# Autodesk Inventor assembly: Slider Assembly
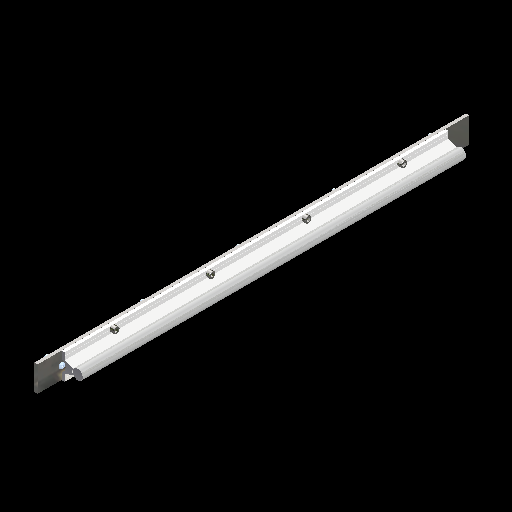
[picture p0: Inventor's stored thumbnail of the model, 512x512]
Saved by Autodesk Inventor 2026.1 (Build 301233000, 233)
## iProperties
Created: 2024-12-30
Part Number: Slider Assembly
Document SubType Name: Assembly
Designer: drago
Author: drago
## Documents named in this file (5)
- C:\Users\drago\Desktop\_QIST4500_Multidisciplinary_Team_Project\Proteox MX magnet positioner CAD\z_rail\z_rail.iam
- C:\Users\drago\Desktop\_QIST4500_Multidisciplinary_Team_Project\Proteox MX magnet positioner CAD\z_rail\item_61953_t-slot-slider-8-80x40-fa__high.ipt
- C:\Users\drago\Desktop\_QIST4500_Multidisciplinary_Team_Project\Proteox MX magnet positioner CAD\z_rail\Rail_bracket.ipt
- C:\Users\drago\Desktop\_QIST4500_Multidisciplinary_Team_Project\Proteox MX magnet positioner CAD\z_rail\SBR16_600mm.ipt
- C:\Users\drago\Documents\Inventor\Content Center Files\R2026\en-US\ISO 4762(2)\ISO 4762 - M6 x 10ISO.ipt
## Components (15 placed, 4 different names)
1. Rail_bracket:1 — Mate:15, Mate:16, Mate:17, Mate:18, Mate:19, Mate:20, Mate:21, Mate:22, Mate:23, Mate:24, Mate:25, Mate:26, Mate:27, Mate:28, Mate:29, Mate:36, Mate:38, Mate:40, Mate:42, Mate:44, Mate:46, Mate:48, Mate:50
2. SBR16_600mm:1 — Mate:16, Mate:17, Mate:18, Mate:37, Mate:39, Mate:41, Mate:43, Mate:45, Mate:47, Mate:49, Mate:51
3. item_61953_t-slot-slider-8-80x40-fa__high:1 — Mate:20, Mate:21, Angle:1
4. item_61953_t-slot-slider-8-80x40-fa__high:2 — Mate:24, Mate:28, Angle:2
5. item_61953_t-slot-slider-8-80x40-fa__high:3 — Mate:22, Mate:26, Angle:3
6. item_61953_t-slot-slider-8-80x40-fa__high:4 — Mate:23, Mate:27, Angle:4
7. item_61953_t-slot-slider-8-80x40-fa__high:5 — Mate:25, Mate:29, Angle:5
8. ISO 4762 M6 x 10:1 — Mate:36, Mate:37
9. ISO 4762 M6 x 10:2 — Mate:38, Mate:39
10. ISO 4762 M6 x 10:3 — Mate:40, Mate:41
11. ISO 4762 M6 x 10:4 — Mate:42, Mate:43
12. ISO 4762 M6 x 10:5 — Mate:44, Mate:45
13. ISO 4762 M6 x 10:6 — Mate:46, Mate:47
14. ISO 4762 M6 x 10:7 — Mate:48, Mate:49
15. ISO 4762 M6 x 10:8 — Mate:50, Mate:51
## Relationships (36: Mate 31, Angle 5)
- Mate:15: Rail_bracket:1
- Mate:16: Rail_bracket:1 ↔ SBR16_600mm:1
- Mate:17: Rail_bracket:1 ↔ SBR16_600mm:1
- Mate:18: Rail_bracket:1 ↔ SBR16_600mm:1
- Mate:19: Rail_bracket:1
- Mate:20: Rail_bracket:1 ↔ item_61953_t-slot-slider-8-80x40-fa__high:1
- Mate:21: Rail_bracket:1 ↔ item_61953_t-slot-slider-8-80x40-fa__high:1
- Angle:1 (0 deg): item_61953_t-slot-slider-8-80x40-fa__high:1
- Mate:22: Rail_bracket:1 ↔ item_61953_t-slot-slider-8-80x40-fa__high:3
- Mate:23: Rail_bracket:1 ↔ item_61953_t-slot-slider-8-80x40-fa__high:4
- Mate:24: Rail_bracket:1 ↔ item_61953_t-slot-slider-8-80x40-fa__high:2
- Mate:25: Rail_bracket:1 ↔ item_61953_t-slot-slider-8-80x40-fa__high:5
- Mate:26: Rail_bracket:1 ↔ item_61953_t-slot-slider-8-80x40-fa__high:3
- Mate:27: Rail_bracket:1 ↔ item_61953_t-slot-slider-8-80x40-fa__high:4
- Mate:28: Rail_bracket:1 ↔ item_61953_t-slot-slider-8-80x40-fa__high:2
- Mate:29: Rail_bracket:1 ↔ item_61953_t-slot-slider-8-80x40-fa__high:5
- Angle:2 (0 deg): item_61953_t-slot-slider-8-80x40-fa__high:2
- Angle:3 (0 deg): item_61953_t-slot-slider-8-80x40-fa__high:3
- Angle:4 (0 deg): item_61953_t-slot-slider-8-80x40-fa__high:4
- Angle:5 (0 deg): item_61953_t-slot-slider-8-80x40-fa__high:5
- Mate:36: Rail_bracket:1 ↔ ISO 4762 M6 x 10:1
- Mate:37: SBR16_600mm:1 ↔ ISO 4762 M6 x 10:1
- Mate:38: Rail_bracket:1 ↔ ISO 4762 M6 x 10:2
- Mate:39: SBR16_600mm:1 ↔ ISO 4762 M6 x 10:2
- Mate:40: Rail_bracket:1 ↔ ISO 4762 M6 x 10:3
- Mate:41: SBR16_600mm:1 ↔ ISO 4762 M6 x 10:3
- Mate:42: Rail_bracket:1 ↔ ISO 4762 M6 x 10:4
- Mate:43: SBR16_600mm:1 ↔ ISO 4762 M6 x 10:4
- Mate:44: Rail_bracket:1 ↔ ISO 4762 M6 x 10:5
- Mate:45: SBR16_600mm:1 ↔ ISO 4762 M6 x 10:5
- Mate:46: Rail_bracket:1 ↔ ISO 4762 M6 x 10:6
- Mate:47: SBR16_600mm:1 ↔ ISO 4762 M6 x 10:6
- Mate:48: Rail_bracket:1 ↔ ISO 4762 M6 x 10:7
- Mate:49: SBR16_600mm:1 ↔ ISO 4762 M6 x 10:7
- Mate:50: Rail_bracket:1 ↔ ISO 4762 M6 x 10:8
- Mate:51: SBR16_600mm:1 ↔ ISO 4762 M6 x 10:8
